# Autodesk Inventor assembly: 61weller
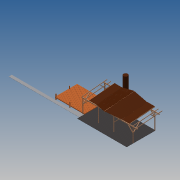
[picture p0: Inventor's stored thumbnail of the model, 180x180]
Saved by Autodesk Inventor 2013 (Build 170138000, 138)
## iProperties
Created: 2014-01-02
Part Number: 61weller
Document SubType Name: Assembly
Designer: ddeboer
Author: ddeboer
## Documents named in this file (13)
- C:\Users\ddeboer\Desktop\house-cad\61weller.iam
- C:\Users\ddeboer\Desktop\house-cad\plat.ipt
- C:\Users\ddeboer\Desktop\house-cad\patio.iam
- C:\Users\ddeboer\Desktop\house-cad\sidewalkBack.ipt
- C:\Users\ddeboer\Desktop\house-cad\2by4by16.ipt
- C:\Users\ddeboer\Desktop\house-cad\tree.ipt
- C:\Users\ddeboer\Desktop\house-cad\wrapAround.ipt
- C:\Users\ddeboer\Desktop\house-cad\bench.ipt
- C:\Users\ddeboer\Desktop\house-cad\planter.ipt
- C:\Users\ddeboer\Desktop\house-cad\2by4by146p5.ipt
- C:\Users\ddeboer\Desktop\house-cad\4by4by34.ipt
- C:\Users\ddeboer\Desktop\house-cad\4by4by17.ipt
- C:\Users\ddeboer\Desktop\house-cad\2by4by18.ipt
## Components (95 placed, 12 different names)
1. plat:1 — Insert:1
2. patio:1 [sub-assembly] — Insert:1, Mate:1, Flush:1, Mate:2, Mate:5, Flush:5, Mate:9, Mate:10, Mate:11, Mate:12, Mate:13
3. sidewalkBack:1 — Mate:1, Flush:1
4. tree:1 — Mate:5, Flush:5
5. wrapAround:1 — Mate:8, Flush:10, Flush:11
6. bench:1
7. planter:1 — Mate:8, Flush:10, Flush:11
8. 2by4by16:10 — Mate:9, Mate:10, Mate:11, Mate:14, Mate:26, Mate:28, Mate:29
9. 2by4by146p5:1 — Mate:14, Flush:12, Flush:13, Mate:18, Mate:20, Flush:18, Mate:23, Mate:27, Flush:26, Flush:27
10. 2by4by146p5:2 — Mate:15, Flush:14, Flush:15, Mate:19, Mate:31
11. 4by4by34:1 — Mate:16, Flush:16, Mate:18
12. 4by4by34:2 — Mate:17, Flush:17, Mate:19, Flush:20
13. 4by4by34:3 — Mate:20, Flush:18, Mate:21
14. 4by4by17:1 — Mate:22, Mate:23, Flush:19
15. 4by4by17:2 — Mate:26, Flush:24, Flush:25
16. 4by4by17:3 — Mate:24, Flush:20, Flush:21, Flush:22
17. 4by4by17:4 — Mate:25, Flush:22, Flush:23, Flush:24
18. 4by4by17:5 — Mate:27, Mate:28, Flush:26
19. 2by4by16:1 — Mate:2, Mate:12, Mate:13, Flush:12, Flush:13, Flush:14, Mate:16, Flush:16, Mate:17, Flush:17, Flush:28, Mate:30, Flush:29
20. 2by4by16:11 — Flush:15
21. 2by4by16:12 — Mate:15
22. 2by4by16:13 — Mate:22, Flush:19, Mate:24, Flush:21
23. 2by4by16:14
24. 2by4by16:15 — Mate:21, Mate:25, Flush:23
25. 2by4by16:16
26. 2by4by16:17 — Flush:25
27. 2by4by146p5:3 — Mate:29, Flush:27, Flush:28
28. 2by4by146p5:4
29. 2by4by146p5:5
30. 2by4by146p5:6
31. 2by4by146p5:7
32. 2by4by146p5:8
33. 2by4by146p5:9
34. 2by4by146p5:10
35. 2by4by146p5:11
36. 2by4by146p5:12
37. 2by4by146p5:13
38. 2by4by146p5:14
39. 2by4by146p5:15
40. 2by4by146p5:16
41. 2by4by146p5:17
42. 2by4by146p5:18
43. 2by4by146p5:19
44. 2by4by146p5:20
45. 2by4by146p5:21
46. 2by4by146p5:22
47. 2by4by146p5:23
48. 2by4by146p5:24
49. 2by4by146p5:25
50. 2by4by146p5:26
51. 2by4by146p5:27
52. 2by4by146p5:28
53. 2by4by146p5:29
54. 2by4by146p5:30
55. 2by4by146p5:31
56. 2by4by146p5:32
57. 2by4by146p5:33
58. 2by4by146p5:34
59. 2by4by146p5:35
60. 2by4by146p5:36
61. 2by4by146p5:37
62. 2by4by146p5:38
63. 2by4by146p5:39
64. 2by4by146p5:40
65. 2by4by146p5:41
66. 2by4by146p5:42
67. 2by4by146p5:43
68. 2by4by146p5:44
69. 2by4by146p5:45
70. 2by4by146p5:46
71. 2by4by146p5:47
72. 2by4by146p5:48
73. 2by4by146p5:49
74. 2by4by146p5:50
75. 2by4by146p5:51
76. 2by4by146p5:52
77. 2by4by146p5:53
78. 2by4by146p5:54
79. 2by4by146p5:55
80. 2by4by18:1 — Mate:30, Flush:29, Mate:31
81. 2by4by18:2
82. 2by4by18:3
83. 2by4by18:4
84. 2by4by18:5
85. 2by4by18:6
86. 2by4by18:7
87. 2by4by18:8
88. 2by4by18:9
89. 2by4by18:10
90. 2by4by18:11
91. 2by4by18:12
92. 2by4by18:13
93. 2by4by18:14
94. 2by4by18:15
95. 2by4by18:16
## Component patterns: (8 elements, first: 2by4by16:1), (53 elements, first: 2by4by146p5:3), (16 elements, first: 2by4by18:1)
## Relationships (50: Mate 27, Flush 22, Insert 1)
- Insert:1: plat:1 ↔ patio:1
- Mate:1: patio:1 ↔ sidewalkBack:1
- Flush:1 (-355.6 mm): patio:1 ↔ sidewalkBack:1
- Mate:2: patio:1 ↔ 2by4by16:1
- Mate:5 (1524 mm): patio:1 ↔ tree:1
- Flush:5 (1016 mm): patio:1 ↔ tree:1
- Mate:8: wrapAround:1 ↔ planter:1
- Flush:10: wrapAround:1 ↔ planter:1
- Flush:11: wrapAround:1 ↔ planter:1
- Mate:9: patio:1 ↔ 2by4by16:10
- Mate:10: patio:1 ↔ 2by4by16:10
- Mate:11: patio:1 ↔ 2by4by16:10
- Mate:12: patio:1 ↔ 2by4by16:1
- Mate:13: patio:1 ↔ 2by4by16:1
- Mate:14: 2by4by16:10 ↔ 2by4by146p5:1
- Flush:12: 2by4by146p5:1 ↔ 2by4by16:1
- Flush:13: 2by4by146p5:1 ↔ 2by4by16:1
- Mate:15: 2by4by146p5:2 ↔ 2by4by16:12
- Flush:14: 2by4by146p5:2 ↔ 2by4by16:1
- Flush:15: 2by4by146p5:2 ↔ 2by4by16:11
- Mate:16: 4by4by34:1 ↔ 2by4by16:1
- Flush:16 (-304.8 mm): 4by4by34:1 ↔ 2by4by16:1
- Mate:17: 4by4by34:2 ↔ 2by4by16:1
- Flush:17 (-304.8 mm): 4by4by34:2 ↔ 2by4by16:1
- Mate:18: 2by4by146p5:1 ↔ 4by4by34:1
- Mate:19 (2438.4 mm): 2by4by146p5:2 ↔ 4by4by34:2
- Mate:20: 2by4by146p5:1 ↔ 4by4by34:3
- Flush:18 (-304.8 mm): 2by4by146p5:1 ↔ 4by4by34:3
- Mate:21: 4by4by34:3 ↔ 2by4by16:15
- Mate:22: 4by4by17:1 ↔ 2by4by16:13
- Mate:23: 2by4by146p5:1 ↔ 4by4by17:1
- Flush:19 (-355.6 mm): 4by4by17:1 ↔ 2by4by16:13
- Mate:24: 4by4by17:3 ↔ 2by4by16:13
- Flush:20: 4by4by34:2 ↔ 4by4by17:3
- Flush:21 (-355.6 mm): 4by4by17:3 ↔ 2by4by16:13
- Mate:25: 4by4by17:4 ↔ 2by4by16:15
- Flush:22: 4by4by17:3 ↔ 4by4by17:4
- Flush:23 (-355.6 mm): 4by4by17:4 ↔ 2by4by16:15
- Mate:26: 2by4by16:10 ↔ 4by4by17:2
- Flush:24: 4by4by17:2 ↔ 4by4by17:4
- Flush:25 (-355.6 mm): 4by4by17:2 ↔ 2by4by16:17
- Mate:27: 2by4by146p5:1 ↔ 4by4by17:5
- Mate:28: 2by4by16:10 ↔ 4by4by17:5
- Flush:26 (-355.6 mm): 2by4by146p5:1 ↔ 4by4by17:5
- Mate:29: 2by4by16:10 ↔ 2by4by146p5:3
- Flush:27: 2by4by146p5:1 ↔ 2by4by146p5:3
- Flush:28: 2by4by16:1 ↔ 2by4by146p5:3
- Mate:30: 2by4by16:1 ↔ 2by4by18:1
- Flush:29: 2by4by16:1 ↔ 2by4by18:1
- Mate:31 (1524 mm): 2by4by146p5:2 ↔ 2by4by18:1
